# Autodesk Inventor assembly: LowerBody
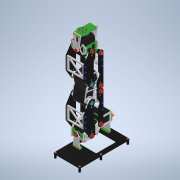
[picture p0: Inventor's stored thumbnail of the model, 180x180]
Saved by Autodesk Inventor 2020.4 (Build 244396000, 396)
## iProperties
Created: 2021-12-27
Part Number: LowerBody
Document SubType Name: Assembly
Designer: Masato Kubotera
Mass: 730.09 g
Surface Area: 2737.95 cm^2
Volume: 452.863 cm^3
Density: 1.61217 g/cm^3
Author: Masato Kubotera
## Documents named in this file (12)
- C:\Users\Masato\Documents\Inventor\CIT Brains_Inventor\OpenPlatform_ver3_0\LowerBody\LowerBody.iam
- C:\Users\Masato\Documents\Inventor\CIT Brains_Inventor\OpenPlatform_ver3_0\LowerBody\Ankle\Ankle.iam
- C:\Users\Masato\Documents\Inventor\CIT Brains_Inventor\OpenPlatform_ver3_0\LowerBody\Ankle\Ankle_side_pitch.iam
- C:\Users\Masato\Documents\Inventor\CIT Brains_Inventor\OpenPlatform_ver3_0\LowerBody\Knee\Knee.iam
- C:\Users\Masato\Documents\Inventor\CIT Brains_Inventor\OpenPlatform_ver3_0\LowerBody\Leg_joit\Leg_joint_roll_pitch.iam
- C:\Users\Masato\Documents\Inventor\CIT Brains_Inventor\OpenPlatform_ver3_0\LowerBody\Leg_joit\Leg_joint_roll_yaw.iam
- C:\Users\Masato\Documents\Inventor\CIT Brains_Inventor\OpenPlatform_ver3_0\LowerBody\Link\BackLowerLink.iam
- C:\Users\Masato\Documents\Inventor\CIT Brains_Inventor\OpenPlatform_ver3_0\LowerBody\Link\BackUpperLink.iam
- C:\Users\Masato\Documents\Inventor\CIT Brains_Inventor\OpenPlatform_ver3_0\LowerBody\Link\FrontLink.iam
- C:\Users\Masato\Documents\Inventor\CIT Brains_Inventor\OpenPlatform_ver3_0\LowerBody\Slider_crank\Slider_crank_mechanism.iam
- C:\Users\Masato\Documents\Inventor\CIT Brains_Inventor\OpenPlatform_ver3_0\ReadyMade\Screw\M2_6-8.ipt
- C:\Users\Masato\Documents\Inventor\CIT Brains_Inventor\OpenPlatform_ver3_0\LowerBody\Foot\Foot.iam
## Components (20 placed, 11 different names)
1. Leg_joint_roll_yaw:1 [sub-assembly] — フラッシュ:1, メイト:1, フラッシュ:2, 挿入:1, 挿入:2, 角度:【付け根ロール軸】, 角度:2
2. Leg_joint_roll_pitch:1 [sub-assembly] — 挿入:1, 挿入:2, 角度:【付け根ロール軸】, 挿入:3, 挿入:4, 挿入:5, 挿入:6, 挿入:7
3. Slider_crank_mechanism:1 [sub-assembly] — 挿入:3, 角度:2
4. FrontLink:1 [sub-assembly] — 挿入:4, 角度:3, 角度:【膝上ピッチ軸】, 挿入:6, 挿入:20
5. BackUpperLink:1 [sub-assembly] — 挿入:5, 角度:3, 挿入:7, 挿入:21
6. Knee:1 [sub-assembly] — 挿入:20, 挿入:21, 挿入:22, 挿入:23, 角度:【膝上ピッチ軸】, 角度:【膝下ピッチ軸】
7. FrontLink:2 [sub-assembly] — 角度:4, 角度:【膝下ピッチ軸】, 挿入:8, 挿入:10, 挿入:22
8. BackLowerLink:1 [sub-assembly] — 角度:4, 挿入:9, 挿入:11, 挿入:23
9. Ankle_side_pitch:1 [sub-assembly] — 挿入:8, 挿入:9, 挿入:12, 挿入:13, 挿入:14, 挿入:15, 挿入:24, 角度:【足首ピッチ軸】
10. Ankle_side_pitch:2 [sub-assembly] — 挿入:10, 挿入:11, 挿入:16, 挿入:17, 挿入:18, 挿入:19
11. Ankle:1 [sub-assembly] — 挿入:24, 角度:【足首ピッチ軸】, 角度:【足首ロール軸】, 挿入:37
12. Foot:1 [sub-assembly] — 角度:【足首ロール軸】, 挿入:37
13. M2_6-8:8 — 挿入:19
14. M2_6-8:7 — 挿入:18
15. M2_6-8:6 — 挿入:17
16. M2_6-8:5 — 挿入:16
17. M2_6-8:4 — 挿入:15
18. M2_6-8:3 — 挿入:14
19. M2_6-8:2 — 挿入:13
20. M2_6-8:1 — 挿入:12
## Relationships (36: Insert 25, Angle 8, Flush 2, Mate 1)
- 角度:【付け根ロール軸】 [Angle] (0 deg): Leg_joint_roll_yaw:1 ↔ Leg_joint_roll_pitch:1
- 角度:【膝上ピッチ軸】 [Angle] (180 deg): FrontLink:1 ↔ Knee:1
- 角度:【膝下ピッチ軸】 [Angle] (0 deg): Knee:1 ↔ FrontLink:2
- 角度:【足首ピッチ軸】 [Angle] (0 deg): Ankle_side_pitch:1 ↔ Ankle:1
- 角度:【足首ロール軸】 [Angle] (0 deg): Ankle:1 ↔ Foot:1
- フラッシュ:1 [Flush]: Leg_joint_roll_yaw:1
- メイト:1 [Mate]: Leg_joint_roll_yaw:1
- フラッシュ:2 [Flush]: Leg_joint_roll_yaw:1
- 挿入:1 [Insert]: Leg_joint_roll_yaw:1 ↔ Leg_joint_roll_pitch:1
- 挿入:2 [Insert]: Leg_joint_roll_yaw:1 ↔ Leg_joint_roll_pitch:1
- 挿入:3 [Insert]: Leg_joint_roll_pitch:1 ↔ Slider_crank_mechanism:1
- 角度:2 [Angle] (0 deg): Leg_joint_roll_yaw:1 ↔ Slider_crank_mechanism:1
- 挿入:4 [Insert]: Leg_joint_roll_pitch:1 ↔ FrontLink:1
- 挿入:5 [Insert]: Leg_joint_roll_pitch:1 ↔ BackUpperLink:1
- 角度:3 [Angle] (0 deg): FrontLink:1 ↔ BackUpperLink:1
- 挿入:6 [Insert]: Leg_joint_roll_pitch:1 ↔ FrontLink:1
- 挿入:7 [Insert]: Leg_joint_roll_pitch:1 ↔ BackUpperLink:1
- 角度:4 [Angle] (0 deg): FrontLink:2 ↔ BackLowerLink:1
- 挿入:8 [Insert]: FrontLink:2 ↔ Ankle_side_pitch:1
- 挿入:9 [Insert]: BackLowerLink:1 ↔ Ankle_side_pitch:1
- 挿入:10 [Insert]: FrontLink:2 ↔ Ankle_side_pitch:2
- 挿入:11 [Insert]: BackLowerLink:1 ↔ Ankle_side_pitch:2
- 挿入:12 [Insert]: Ankle_side_pitch:1 ↔ M2_6-8:1
- 挿入:13 [Insert]: Ankle_side_pitch:1 ↔ M2_6-8:2
- 挿入:14 [Insert]: Ankle_side_pitch:1 ↔ M2_6-8:3
- 挿入:15 [Insert]: Ankle_side_pitch:1 ↔ M2_6-8:4
- 挿入:16 [Insert]: Ankle_side_pitch:2 ↔ M2_6-8:5
- 挿入:17 [Insert]: Ankle_side_pitch:2 ↔ M2_6-8:6
- 挿入:18 [Insert]: Ankle_side_pitch:2 ↔ M2_6-8:7
- 挿入:19 [Insert]: Ankle_side_pitch:2 ↔ M2_6-8:8
- 挿入:20 [Insert]: FrontLink:1 ↔ Knee:1
- 挿入:21 [Insert]: BackUpperLink:1 ↔ Knee:1
- 挿入:22 [Insert]: Knee:1 ↔ FrontLink:2
- 挿入:23 [Insert]: Knee:1 ↔ BackLowerLink:1
- 挿入:24 [Insert]: Ankle_side_pitch:1 ↔ Ankle:1
- 挿入:37 [Insert]: Ankle:1 ↔ Foot:1
